# Autodesk Inventor assembly: am-0940
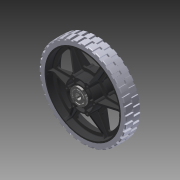
[picture p0: Inventor's stored thumbnail of the model, 180x180]
Saved by Autodesk Inventor 2013 (Build 170138000, 138)
## iProperties
Category: Drive Base Kit
Company: Autodesk Inc.
Created: 2012-12-27
Part Number: am-0940
Document SubType Name: Assembly
Designer: Autodesk Inc.
Catalog Web Link: http://www.andymark.com/product-p/am-0940.htm
Vendor: AndyMark Inc.
Mass: 226.796 g
Surface Area: 1150.49 cm^2
Volume: 196.611 cm^3
Author: Autodesk Inc.
## Documents named in this file (4)
- E:\Data Folder\FIRST 2013\FIRST KOP\Parts\Drive Base Kit\DBK_HiGripWheel_am-0940.iam
- E:\Data Folder\FIRST 2013\FIRST KOP\Parts\Drive Base Kit\6 HiGrip Tread.ipt
- E:\Data Folder\FIRST 2013\FIRST KOP\Parts\Drive Base Kit\6in 2008 FIRST Hub.ipt
- E:\Data Folder\FIRST 2013\FIRST KOP\Parts\Drive Base Kit\DBK_1614ZZBearing_am-0209.ipt
## Components (4 placed, 3 different names)
1. 6 HiGrip Tread:1
2. 6in 2008 FIRST Hub:1 — Insert:1, Insert:2
3. DBK_1614ZZBearing_am-0209:1 — Insert:2
4. DBK_1614ZZBearing_am-0209:2 — Insert:1
## Relationships (2: Insert 2)
- Insert:1: 6in 2008 FIRST Hub:1 ↔ DBK_1614ZZBearing_am-0209:2
- Insert:2: 6in 2008 FIRST Hub:1 ↔ DBK_1614ZZBearing_am-0209:1
